# Autodesk Inventor assembly: FrameV3
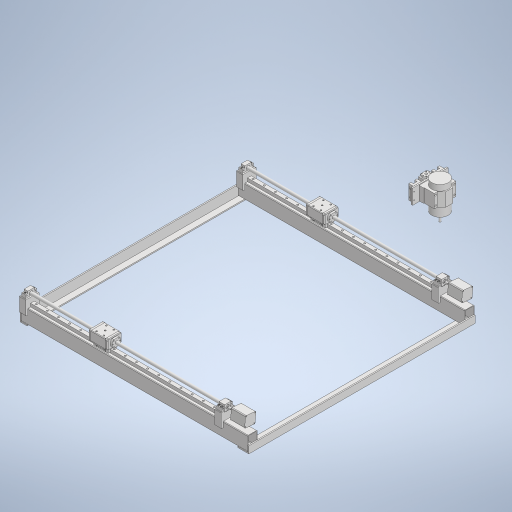
[picture p0: Inventor's stored thumbnail of the model, 512x512]
Saved by Autodesk Inventor 2023 (Build 270158000, 158)
## iProperties
Created: 2022-05-03
Part Number: FrameV3
Document SubType Name: Assembly
Designer: plebbb
Author: plebbb
## Documents named in this file (13)
- D:\Users\plebbb\Desktop\CNC_Project\FrameV3.iam
- D:\Users\plebbb\Desktop\CNC_Project\Ballscrew_Assembly.iam
- D:\Users\plebbb\Desktop\CNC_Project\X_GANTRY.iam
- D:\Users\plebbb\Desktop\CNC_Project\Steel_L_Bracket.ipt
- D:\Users\plebbb\Desktop\CNC_Project\Spindle.ipt
- D:\Users\plebbb\Desktop\CNC_Project\Spindle_Holder.ipt
- D:\Users\plebbb\Desktop\CNC_Project\Z_PLATE.iam
- D:\Users\plebbb\Desktop\CNC_Project\FrameV3\AIP\FEA\dyol7vh0g.fins
- D:\Users\plebbb\Desktop\CNC_Project\FrameV3\AIP\FEA\dyol7vh0g.fsat
- D:\Users\plebbb\Desktop\CNC_Project\FrameV3\AIP\FEA\dyol7vh0g.ftes
- D:\Users\plebbb\Desktop\CNC_Project\FrameV3\AIP\FEA\dyol7vh0g.fwiz
- D:\Users\plebbb\Desktop\CNC_Project\FrameV3\AIP\FEA\dyol7vheo.fmsh
- D:\Users\plebbb\Desktop\CNC_Project\FrameV3\AIP\FEA\dyol7vhep.fres
## Components (9 placed, 6 different names)
1. Ballscrew_Assembly:1 [sub-assembly]
2. X_GANTRY:1 [sub-assembly] — Mate:30, Mate:31, Flush:4, Mate:38, Flush:9, Mate:40, Flush:49
3. X_GANTRY:2 [sub-assembly] — Mate:25, Mate:26, Mate:27, Mate:28, Mate:29, Mate:34, Mate:37, Flush:6, Mate:39, Flush:8
4. Ballscrew_Assembly:2 [sub-assembly] — Mate:25, Mate:26, Mate:27, Mate:28, Mate:29
5. Steel_L_Bracket:1 — Mate:30, Mate:31, Flush:4, Mate:34, Mate:37, Flush:6, Flush:42, Mate:42, Mate:69
6. Steel_L_Bracket:3 — Mate:38, Mate:39, Flush:8, Flush:9, Mate:40
7. Spindle:1 — Mate:70, Flush:43, Flush:49
8. Spindle_Holder:1 — Mate:70, Flush:43
9. Z_PLATE:1 [sub-assembly]
## Relationships (33: Mate 24, Flush 9)
- [Mate]: Ballscrew_Assembly:1 ↔ X_GANTRY:1
- [Mate]: Ballscrew_Assembly:1 ↔ X_GANTRY:1
- [Flush]: Ballscrew_Assembly:1 ↔ X_GANTRY:1
- [Flush]: Ballscrew_Assembly:1 ↔ X_GANTRY:1
- [Mate]: Ballscrew_Assembly:1 ↔ X_GANTRY:1
- [Mate]: Ballscrew_Assembly:1 ↔ X_GANTRY:1
- [Mate]: Ballscrew_Assembly:1 ↔ X_GANTRY:1
- [Mate]: Ballscrew_Assembly:1 ↔ X_GANTRY:1
- Mate:25: X_GANTRY:2 ↔ Ballscrew_Assembly:2
- Mate:26: X_GANTRY:2 ↔ Ballscrew_Assembly:2
- Mate:27: X_GANTRY:2 ↔ Ballscrew_Assembly:2
- Mate:28: X_GANTRY:2 ↔ Ballscrew_Assembly:2
- Mate:29: X_GANTRY:2 ↔ Ballscrew_Assembly:2
- Mate:30: X_GANTRY:1 ↔ Steel_L_Bracket:1
- Mate:31: X_GANTRY:1 ↔ Steel_L_Bracket:1
- Flush:4: X_GANTRY:1 ↔ Steel_L_Bracket:1
- Mate:34: X_GANTRY:2 ↔ Steel_L_Bracket:1
- Mate:37: X_GANTRY:2 ↔ Steel_L_Bracket:1
- Flush:6: X_GANTRY:2 ↔ Steel_L_Bracket:1
- Mate:38: X_GANTRY:1 ↔ Steel_L_Bracket:3
- Mate:39: X_GANTRY:2 ↔ Steel_L_Bracket:3
- Flush:8: X_GANTRY:2 ↔ Steel_L_Bracket:3
- Flush:9: X_GANTRY:1 ↔ Steel_L_Bracket:3
- Mate:40: X_GANTRY:1 ↔ Steel_L_Bracket:3
- Flush:42: Steel_L_Bracket:1
- Mate:42: Steel_L_Bracket:1
- Mate:69: Steel_L_Bracket:1
- Mate:70: Spindle:1 ↔ Spindle_Holder:1
- Flush:43 (50 mm): Spindle:1 ↔ Spindle_Holder:1
- [Mate]: Spindle_Holder:1 ↔ Z_PLATE:1
- [Mate]: Spindle_Holder:1 ↔ Z_PLATE:1
- [Mate]: Spindle_Holder:1 ↔ Z_PLATE:1
- Flush:49: X_GANTRY:1 ↔ Spindle:1
## Named parameters: sa_0 = 100000
note: some values were not read from the file. Shown as the stored number, unit unknown: "sa_0".
